# Autodesk Inventor assembly: Handle Hafele 115.70 on Facade
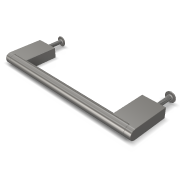
[picture p0: Inventor's stored thumbnail of the model, 180x180]
Saved by Autodesk Inventor 2024 (Build 280153000, 153)
## iProperties
RuleStatus: InUse
Created: 2023-02-20
Part Number: Handle Hafele 115.70 on Facade
Document SubType Name: Assembly
Designer: sauliusd
Author: sauliusd
## Documents named in this file (3)
- C:\W4INV 2024 Design\SMART HARDWARE\Handles\Hafele Handle 115.70\Handle Hafele 115.70 on Facade.iam
- C:\W4INV 2024 Design\SMART HARDWARE\Handles\Hafele Handle 115.70\Parts\Hafele Handle 115.70 Skeleton.ipt
- C:\W4INV 2024 Design\SMART HARDWARE\Handles\Hafele Handle 115.70\Parts\Hafele Handle 115.70.iam
## Components (2 placed, 2 different names)
1. @Skeleton — Flush:1, Flush:2, Flush:3, Mate:1, Flush:4
2. Hafele Handle 115.70 [sub-assembly] — Mate:1, Flush:4
## Relationships (5: Flush 4, Mate 1)
- Flush:1: @Skeleton
- Flush:2: @Skeleton
- Flush:3: @Skeleton
- Mate:1: @Skeleton ↔ Hafele Handle 115.70
- Flush:4: @Skeleton ↔ Hafele Handle 115.70
## Named parameters: HandleLength = 148 mm, FacadeWidth = 400 mm, FacadeHeight = 700 mm, DistFromSide_X = 50 mm, DistFromSide_Y = 60 mm, FacadeThickness = 18 mm
